# Autodesk Inventor assembly: Foot2Assembly
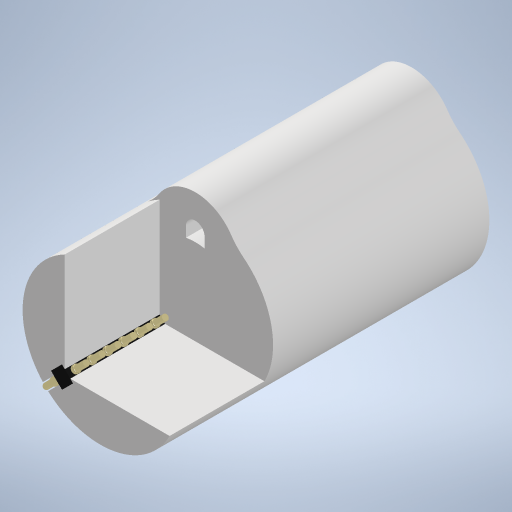
[picture p0: Inventor's stored thumbnail of the model, 512x512]
Saved by Autodesk Inventor 2023 (Build 270158000, 158)
## iProperties
Created: 2023-01-25
Part Number: Foot2Assembly
Document SubType Name: Assembly
Designer: chase
Author: chase
## Documents named in this file (3)
- C:\Users\chase\OneDrive\Documents\GitHub\WU-Team20-AutonomousDrone\CAD\Legs\Foot2Assembly.iam
- C:\Users\chase\OneDrive\Documents\GitHub\WU-Team20-AutonomousDrone\CAD\Legs\LandingFoot2.ipt
- C:\Users\chase\OneDrive\Documents\GitHub\WU-Team20-AutonomousDrone\CAD\Legs\PogoPins - 1x6Array.ipt
## Components (2 placed, 2 different names)
1. LandingFoot2:1 — Mate:1, Mate:2, Mate:3
2. PogoPins - 1x6Array:1 — Mate:1, Mate:2, Mate:3
## Relationships (3: Mate 3)
- Mate:1: LandingFoot2:1 ↔ PogoPins - 1x6Array:1
- Mate:2: LandingFoot2:1 ↔ PogoPins - 1x6Array:1
- Mate:3: LandingFoot2:1 ↔ PogoPins - 1x6Array:1
